# Autodesk Inventor assembly: box
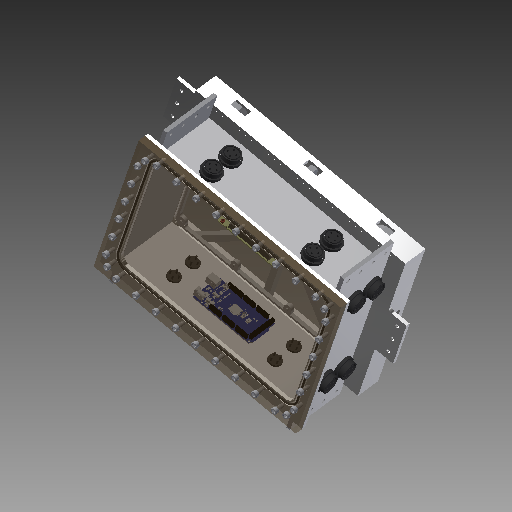
[picture p0: Inventor's stored thumbnail of the model, 512x512]
Saved by Autodesk Inventor 2018.1 (Build 221171000, 171)
## iProperties
Created: 2017-08-02
Part Number: box
Document SubType Name: Assembly
Designer: Kai
Author: Kai
## Documents named in this file (19)
- E:\robosub\box.iam
- E:\robosub\longsides.ipt
- E:\robosub\shortsides.ipt
- E:\robosub\smallgasketback.ipt
- E:\robosub\91292A137_TYPE 18-8 SS SOCKET HEAD CAP SCREW.ipt
- E:\robosub\top.ipt
- E:\robosub\toppoly.ipt
- E:\robosub\bottom3.ipt
- E:\robosub\alumbottom3.ipt
- E:\robosub\pin holder.ipt
- E:\robosub\pins.ipt
- E:\robosub\91292A134_TYPE 18-8 SS SOCKET HEAD CAP SCREW.ipt
- E:\robosub\lid guide.ipt
- E:\robosub\99397A074_METRIC THREAD-FORMING SCREW FOR PLASTICS.ipt
- E:\robosub\latchplate.ipt
- E:\robosub\latchplate2.ipt
- E:\robosub\NUC5i3MYBE- GRABCAD.ipt
- E:\robosub\arduino MEGA2650.ipt
- E:\robosub\connector.ipt
## Components (83 placed, 18 different names)
1. longsides:1 — Mate:6, Flush:8, Mate:242, Mate:252, Mate:253, Mate:254, Mate:255, Mate:256, Mate:257, Mate:258, Mate:259, Mate:260
2. longsides:2 — Mate:3, Mate:106, Mate:107, Mate:108, Mate:109, Flush:3, Flush:20, Mate:240, Mate:248, Mate:249, Mate:250, Mate:251, Mate:261, Mate:262, Mate:263, Mate:264
3. shortsides:1 — Mate:3, Mate:106, Mate:108, Flush:9, Mate:116, Mate:239
4. shortsides:2 — Mate:6, Mate:107, Mate:109, Mate:111, Mate:112, Mate:239, Mate:241, Mate:243, Mate:244, Mate:245, Mate:246, Mate:247, Tangent:2, Tangent:3, Tangent:4, Tangent:5, Tangent:6, Tangent:8
5. smallgasketback:1 — Mate:117, Mate:118
6. top:1 — Mate:111, Mate:112, Flush:3, Mate:113, Mate:114, Mate:115, Flush:4, Flush:5, Mate:213, Mate:214, Mate:235, Flush:12, Flush:13, Mate:236, Flush:14, Flush:15, Mate:237, Flush:16, Mate:238, Flush:18
7. smallgasketback:2 — Mate:113, Mate:114
8. toppoly:1 — Mate:115, Flush:4, Flush:5, Mate:193, Flush:10, Flush:11, Mate:212
9. bottom3:1 — Mate:119, Mate:120, Mate:121, Mate:122, Mate:123, Mate:124, Mate:125, Mate:126, Mate:127, Mate:128, Mate:129, Mate:130, Mate:131, Mate:132, Mate:133, Mate:134, Mate:135, Mate:136, Mate:137, Mate:138, Mate:139, Mate:140, Mate:141, Mate:142, Mate:143, Mate:144, Mate:145, Mate:146, Mate:147, Mate:148, Mate:149, Mate:150, Mate:151, Mate:152, Mate:153, Mate:154, Mate:155, Mate:156, Mate:157, Mate:158, Mate:159, Mate:160, Mate:161, Mate:162, Mate:163, Mate:164, Mate:165, Mate:166, Mate:167, Mate:168, Mate:169, Mate:170, Mate:171, Mate:172, Mate:173, Mate:174, Mate:175, Mate:176, Mate:177, Mate:178, Mate:179, Mate:180, Mate:181, Mate:182, Mate:183, Mate:184, Mate:185, Mate:186, Mate:187, Mate:188, Mate:189
10. alumbottom3:1 — Flush:8, Flush:9, Mate:116, Mate:117, Mate:118, Mate:119, Mate:120, Mate:121, Flush:20, Flush:21, Flush:22, Mate:256
11. 91292A137_TYPE 18-8 SS SOCKET HEAD CAP SCREW:1 — Mate:123, Mate:188
12. 91292A137_TYPE 18-8 SS SOCKET HEAD CAP SCREW:2 — Mate:124, Mate:189
13. 91292A137_TYPE 18-8 SS SOCKET HEAD CAP SCREW:3 — Mate:125, Mate:158
14. 91292A137_TYPE 18-8 SS SOCKET HEAD CAP SCREW:4 — Mate:126, Mate:157
15. 91292A137_TYPE 18-8 SS SOCKET HEAD CAP SCREW:5 — Mate:127, Mate:156
16. 91292A137_TYPE 18-8 SS SOCKET HEAD CAP SCREW:6 — Mate:128, Mate:159
17. 91292A137_TYPE 18-8 SS SOCKET HEAD CAP SCREW:7 — Mate:129, Mate:160
18. 91292A137_TYPE 18-8 SS SOCKET HEAD CAP SCREW:8 — Mate:130, Mate:161
19. 91292A137_TYPE 18-8 SS SOCKET HEAD CAP SCREW:9 — Mate:131, Mate:162
20. 91292A137_TYPE 18-8 SS SOCKET HEAD CAP SCREW:10 — Mate:132, Mate:163
21. 91292A137_TYPE 18-8 SS SOCKET HEAD CAP SCREW:11 — Mate:133, Mate:164
22. 91292A137_TYPE 18-8 SS SOCKET HEAD CAP SCREW:12 — Mate:134, Mate:165
23. 91292A137_TYPE 18-8 SS SOCKET HEAD CAP SCREW:13 — Mate:135, Mate:166
24. 91292A137_TYPE 18-8 SS SOCKET HEAD CAP SCREW:14 — Mate:136, Mate:167
25. 91292A137_TYPE 18-8 SS SOCKET HEAD CAP SCREW:15 — Mate:137, Mate:168
26. 91292A137_TYPE 18-8 SS SOCKET HEAD CAP SCREW:16 — Mate:138, Mate:169
27. 91292A137_TYPE 18-8 SS SOCKET HEAD CAP SCREW:17 — Mate:139, Mate:170
28. 91292A137_TYPE 18-8 SS SOCKET HEAD CAP SCREW:18 — Mate:140, Mate:171
29. 91292A137_TYPE 18-8 SS SOCKET HEAD CAP SCREW:19 — Mate:141, Mate:172
30. 91292A137_TYPE 18-8 SS SOCKET HEAD CAP SCREW:20 — Mate:142, Mate:173
31. 91292A137_TYPE 18-8 SS SOCKET HEAD CAP SCREW:21 — Mate:144, Mate:175
32. 91292A137_TYPE 18-8 SS SOCKET HEAD CAP SCREW:22 — Mate:143, Mate:174
33. 91292A137_TYPE 18-8 SS SOCKET HEAD CAP SCREW:23 — Mate:145, Mate:176
34. 91292A137_TYPE 18-8 SS SOCKET HEAD CAP SCREW:24 — Mate:147, Mate:178
35. 91292A137_TYPE 18-8 SS SOCKET HEAD CAP SCREW:25 — Mate:148, Mate:179
36. 91292A137_TYPE 18-8 SS SOCKET HEAD CAP SCREW:26 — Mate:149, Mate:180
37. 91292A137_TYPE 18-8 SS SOCKET HEAD CAP SCREW:27 — Mate:150, Mate:181
38. 91292A137_TYPE 18-8 SS SOCKET HEAD CAP SCREW:28 — Mate:151, Mate:182
39. 91292A137_TYPE 18-8 SS SOCKET HEAD CAP SCREW:29 — Mate:152, Mate:183
40. 91292A137_TYPE 18-8 SS SOCKET HEAD CAP SCREW:30 — Mate:153, Mate:184
41. 91292A137_TYPE 18-8 SS SOCKET HEAD CAP SCREW:31 — Mate:154, Mate:185
42. 91292A137_TYPE 18-8 SS SOCKET HEAD CAP SCREW:32 — Mate:155, Mate:186
43. 91292A137_TYPE 18-8 SS SOCKET HEAD CAP SCREW:33 — Mate:146, Mate:177
44. 91292A137_TYPE 18-8 SS SOCKET HEAD CAP SCREW:34 — Mate:122, Mate:187
45. pin holder:1 — Mate:194, Mate:195
46. pins:1 — Mate:193, Mate:194, Mate:195, Flush:10, Flush:11, Mate:196, Mate:197, Mate:198, Mate:199, Mate:200, Mate:201, Mate:202, Mate:203, Mate:204, Mate:205, Mate:206, Mate:207, Mate:208, Mate:209, Mate:210, Mate:211
47. 91292A134_TYPE 18-8 SS SOCKET HEAD CAP SCREW:1 — Mate:199, Mate:208
48. 91292A134_TYPE 18-8 SS SOCKET HEAD CAP SCREW:2 — Mate:201, Mate:205
49. 91292A134_TYPE 18-8 SS SOCKET HEAD CAP SCREW:3 — Mate:200, Mate:207
50. 91292A134_TYPE 18-8 SS SOCKET HEAD CAP SCREW:4 — Mate:202, Mate:211
51. 91292A134_TYPE 18-8 SS SOCKET HEAD CAP SCREW:5 — Mate:197, Mate:209
52. 91292A134_TYPE 18-8 SS SOCKET HEAD CAP SCREW:6 — Mate:196, Mate:204
53. 91292A134_TYPE 18-8 SS SOCKET HEAD CAP SCREW:7 — Mate:198, Mate:210
54. 91292A134_TYPE 18-8 SS SOCKET HEAD CAP SCREW:8 — Mate:203, Mate:206
55. lid guide:1 — Mate:212, Mate:213, Mate:214, Mate:215, Mate:216, Mate:217, Mate:218, Mate:219, Mate:220, Mate:221, Mate:222, Mate:223, Mate:224, Mate:225, Mate:226, Mate:227, Mate:228, Mate:229, Mate:230, Mate:231, Mate:232, Mate:233, Mate:234
56. 99397A074_METRIC THREAD-FORMING SCREW FOR PLASTICS:1 — Mate:224, Mate:226
57. 99397A074_METRIC THREAD-FORMING SCREW FOR PLASTICS:2 — Mate:215, Mate:231
58. 99397A074_METRIC THREAD-FORMING SCREW FOR PLASTICS:3 — Mate:221, Mate:228
59. 99397A074_METRIC THREAD-FORMING SCREW FOR PLASTICS:4 — Mate:222, Mate:227
60. 99397A074_METRIC THREAD-FORMING SCREW FOR PLASTICS:5 — Mate:217, Mate:230
61. 99397A074_METRIC THREAD-FORMING SCREW FOR PLASTICS:6 — Mate:216, Mate:232
62. 99397A074_METRIC THREAD-FORMING SCREW FOR PLASTICS:7 — Mate:223, Mate:225
63. 99397A074_METRIC THREAD-FORMING SCREW FOR PLASTICS:8 — Mate:219, Mate:229
64. 99397A074_METRIC THREAD-FORMING SCREW FOR PLASTICS:9 — Mate:218, Mate:233
65. 99397A074_METRIC THREAD-FORMING SCREW FOR PLASTICS:10 — Mate:220, Mate:234
66. latchplate:2 — Mate:235, Flush:12, Flush:13
67. latchplate:3 — Mate:236, Flush:14, Flush:15, Flush:17, Flush:19
68. latchplate2:1 — Mate:237, Flush:16, Flush:17, Tangent:1, Tangent:7
69. latchplate2:2 — Mate:238, Flush:18, Flush:19
70. NUC5i3MYBE- GRABCAD:1 — Mate:240, Flush:21, Mate:241
71. arduino MEGA2650:1 — Mate:242, Flush:22, Mate:243
72. connector:1 — Mate:244, Tangent:1, Tangent:2
73. connector:2 — Mate:245, Tangent:7, Tangent:8
74. connector:3 — Mate:246, Tangent:5, Tangent:6
75. connector:4 — Mate:247, Tangent:3, Tangent:4
76. connector:5 — Mate:248, Mate:262
77. connector:6 — Mate:251, Mate:263
78. connector:7 — Mate:249, Mate:264
79. connector:8 — Mate:250, Mate:261
80. connector:9 — Mate:253, Mate:257
81. connector:10 — Mate:255, Mate:259
82. connector:11 — Mate:252, Mate:258
83. connector:12 — Mate:254, Mate:260
## Relationships (183: Mate 157, Flush 18, Tangent 8)
- Mate:3: longsides:2 ↔ shortsides:1
- Mate:6: longsides:1 ↔ shortsides:2
- Mate:106: longsides:2 ↔ shortsides:1
- Mate:107: longsides:2 ↔ shortsides:2
- Mate:108: longsides:2 ↔ shortsides:1
- Mate:109: longsides:2 ↔ shortsides:2
- Mate:111: shortsides:2 ↔ top:1
- Mate:112 (304.8 mm): shortsides:2 ↔ top:1
- Flush:3 (-19.05 mm): longsides:2 ↔ top:1
- Mate:113: top:1 ↔ smallgasketback:2
- Mate:114: top:1 ↔ smallgasketback:2
- Mate:115: top:1 ↔ toppoly:1
- Flush:4: top:1 ↔ toppoly:1
- Flush:5: top:1 ↔ toppoly:1
- Flush:8: longsides:1 ↔ alumbottom3:1
- Flush:9: shortsides:1 ↔ alumbottom3:1
- Mate:116: shortsides:1 ↔ alumbottom3:1
- Mate:117: smallgasketback:1 ↔ alumbottom3:1
- Mate:118: smallgasketback:1 ↔ alumbottom3:1
- Mate:119: bottom3:1 ↔ alumbottom3:1
- Mate:120: bottom3:1 ↔ alumbottom3:1
- Mate:121: bottom3:1 ↔ alumbottom3:1
- Mate:122: bottom3:1 ↔ 91292A137_TYPE 18-8 SS SOCKET HEAD CAP SCREW:34
- Mate:123: bottom3:1 ↔ 91292A137_TYPE 18-8 SS SOCKET HEAD CAP SCREW:1
- Mate:124: bottom3:1 ↔ 91292A137_TYPE 18-8 SS SOCKET HEAD CAP SCREW:2
- Mate:125: bottom3:1 ↔ 91292A137_TYPE 18-8 SS SOCKET HEAD CAP SCREW:3
- Mate:126: bottom3:1 ↔ 91292A137_TYPE 18-8 SS SOCKET HEAD CAP SCREW:4
- Mate:127: bottom3:1 ↔ 91292A137_TYPE 18-8 SS SOCKET HEAD CAP SCREW:5
- Mate:128: bottom3:1 ↔ 91292A137_TYPE 18-8 SS SOCKET HEAD CAP SCREW:6
- Mate:129: bottom3:1 ↔ 91292A137_TYPE 18-8 SS SOCKET HEAD CAP SCREW:7
- Mate:130: bottom3:1 ↔ 91292A137_TYPE 18-8 SS SOCKET HEAD CAP SCREW:8
- Mate:131: bottom3:1 ↔ 91292A137_TYPE 18-8 SS SOCKET HEAD CAP SCREW:9
- Mate:132: bottom3:1 ↔ 91292A137_TYPE 18-8 SS SOCKET HEAD CAP SCREW:10
- Mate:133: bottom3:1 ↔ 91292A137_TYPE 18-8 SS SOCKET HEAD CAP SCREW:11
- Mate:134: bottom3:1 ↔ 91292A137_TYPE 18-8 SS SOCKET HEAD CAP SCREW:12
- Mate:135: bottom3:1 ↔ 91292A137_TYPE 18-8 SS SOCKET HEAD CAP SCREW:13
- Mate:136: bottom3:1 ↔ 91292A137_TYPE 18-8 SS SOCKET HEAD CAP SCREW:14
- Mate:137: bottom3:1 ↔ 91292A137_TYPE 18-8 SS SOCKET HEAD CAP SCREW:15
- Mate:138: bottom3:1 ↔ 91292A137_TYPE 18-8 SS SOCKET HEAD CAP SCREW:16
- Mate:139: bottom3:1 ↔ 91292A137_TYPE 18-8 SS SOCKET HEAD CAP SCREW:17
- Mate:140: bottom3:1 ↔ 91292A137_TYPE 18-8 SS SOCKET HEAD CAP SCREW:18
- Mate:141: bottom3:1 ↔ 91292A137_TYPE 18-8 SS SOCKET HEAD CAP SCREW:19
- Mate:142: bottom3:1 ↔ 91292A137_TYPE 18-8 SS SOCKET HEAD CAP SCREW:20
- Mate:143: bottom3:1 ↔ 91292A137_TYPE 18-8 SS SOCKET HEAD CAP SCREW:22
- Mate:144: bottom3:1 ↔ 91292A137_TYPE 18-8 SS SOCKET HEAD CAP SCREW:21
- Mate:145: bottom3:1 ↔ 91292A137_TYPE 18-8 SS SOCKET HEAD CAP SCREW:23
- Mate:146: bottom3:1 ↔ 91292A137_TYPE 18-8 SS SOCKET HEAD CAP SCREW:33
- Mate:147: bottom3:1 ↔ 91292A137_TYPE 18-8 SS SOCKET HEAD CAP SCREW:24
- Mate:148: bottom3:1 ↔ 91292A137_TYPE 18-8 SS SOCKET HEAD CAP SCREW:25
- Mate:149: bottom3:1 ↔ 91292A137_TYPE 18-8 SS SOCKET HEAD CAP SCREW:26
- Mate:150: bottom3:1 ↔ 91292A137_TYPE 18-8 SS SOCKET HEAD CAP SCREW:27
- Mate:151: bottom3:1 ↔ 91292A137_TYPE 18-8 SS SOCKET HEAD CAP SCREW:28
- Mate:152: bottom3:1 ↔ 91292A137_TYPE 18-8 SS SOCKET HEAD CAP SCREW:29
- Mate:153: bottom3:1 ↔ 91292A137_TYPE 18-8 SS SOCKET HEAD CAP SCREW:30
- Mate:154: bottom3:1 ↔ 91292A137_TYPE 18-8 SS SOCKET HEAD CAP SCREW:31
- Mate:155: bottom3:1 ↔ 91292A137_TYPE 18-8 SS SOCKET HEAD CAP SCREW:32
- Mate:156: bottom3:1 ↔ 91292A137_TYPE 18-8 SS SOCKET HEAD CAP SCREW:5
- Mate:157: bottom3:1 ↔ 91292A137_TYPE 18-8 SS SOCKET HEAD CAP SCREW:4
- Mate:158: bottom3:1 ↔ 91292A137_TYPE 18-8 SS SOCKET HEAD CAP SCREW:3
- Mate:159: bottom3:1 ↔ 91292A137_TYPE 18-8 SS SOCKET HEAD CAP SCREW:6
- Mate:160: bottom3:1 ↔ 91292A137_TYPE 18-8 SS SOCKET HEAD CAP SCREW:7
- Mate:161: bottom3:1 ↔ 91292A137_TYPE 18-8 SS SOCKET HEAD CAP SCREW:8
- Mate:162: bottom3:1 ↔ 91292A137_TYPE 18-8 SS SOCKET HEAD CAP SCREW:9
- Mate:163: bottom3:1 ↔ 91292A137_TYPE 18-8 SS SOCKET HEAD CAP SCREW:10
- Mate:164: bottom3:1 ↔ 91292A137_TYPE 18-8 SS SOCKET HEAD CAP SCREW:11
- Mate:165: bottom3:1 ↔ 91292A137_TYPE 18-8 SS SOCKET HEAD CAP SCREW:12
- Mate:166: bottom3:1 ↔ 91292A137_TYPE 18-8 SS SOCKET HEAD CAP SCREW:13
- Mate:167: bottom3:1 ↔ 91292A137_TYPE 18-8 SS SOCKET HEAD CAP SCREW:14
- Mate:168: bottom3:1 ↔ 91292A137_TYPE 18-8 SS SOCKET HEAD CAP SCREW:15
- Mate:169: bottom3:1 ↔ 91292A137_TYPE 18-8 SS SOCKET HEAD CAP SCREW:16
- Mate:170: bottom3:1 ↔ 91292A137_TYPE 18-8 SS SOCKET HEAD CAP SCREW:17
- Mate:171: bottom3:1 ↔ 91292A137_TYPE 18-8 SS SOCKET HEAD CAP SCREW:18
- Mate:172: bottom3:1 ↔ 91292A137_TYPE 18-8 SS SOCKET HEAD CAP SCREW:19
- Mate:173: bottom3:1 ↔ 91292A137_TYPE 18-8 SS SOCKET HEAD CAP SCREW:20
- Mate:174: bottom3:1 ↔ 91292A137_TYPE 18-8 SS SOCKET HEAD CAP SCREW:22
- Mate:175: bottom3:1 ↔ 91292A137_TYPE 18-8 SS SOCKET HEAD CAP SCREW:21
- Mate:176: bottom3:1 ↔ 91292A137_TYPE 18-8 SS SOCKET HEAD CAP SCREW:23
- Mate:177: bottom3:1 ↔ 91292A137_TYPE 18-8 SS SOCKET HEAD CAP SCREW:33
- Mate:178: bottom3:1 ↔ 91292A137_TYPE 18-8 SS SOCKET HEAD CAP SCREW:24
- Mate:179: bottom3:1 ↔ 91292A137_TYPE 18-8 SS SOCKET HEAD CAP SCREW:25
- Mate:180: bottom3:1 ↔ 91292A137_TYPE 18-8 SS SOCKET HEAD CAP SCREW:26
- Mate:181: bottom3:1 ↔ 91292A137_TYPE 18-8 SS SOCKET HEAD CAP SCREW:27
- Mate:182: bottom3:1 ↔ 91292A137_TYPE 18-8 SS SOCKET HEAD CAP SCREW:28
- Mate:183: bottom3:1 ↔ 91292A137_TYPE 18-8 SS SOCKET HEAD CAP SCREW:29
- Mate:184: bottom3:1 ↔ 91292A137_TYPE 18-8 SS SOCKET HEAD CAP SCREW:30
- Mate:185: bottom3:1 ↔ 91292A137_TYPE 18-8 SS SOCKET HEAD CAP SCREW:31
- Mate:186: bottom3:1 ↔ 91292A137_TYPE 18-8 SS SOCKET HEAD CAP SCREW:32
- Mate:187: bottom3:1 ↔ 91292A137_TYPE 18-8 SS SOCKET HEAD CAP SCREW:34
- Mate:188: bottom3:1 ↔ 91292A137_TYPE 18-8 SS SOCKET HEAD CAP SCREW:1
- Mate:189: bottom3:1 ↔ 91292A137_TYPE 18-8 SS SOCKET HEAD CAP SCREW:2
- Mate:193: toppoly:1 ↔ pins:1
- Mate:194: pin holder:1 ↔ pins:1
- Mate:195: pin holder:1 ↔ pins:1
- Flush:10 (-6.35 mm): toppoly:1 ↔ pins:1
- Flush:11 (-6.35 mm): toppoly:1 ↔ pins:1
- Mate:196: pins:1 ↔ 91292A134_TYPE 18-8 SS SOCKET HEAD CAP SCREW:6
- Mate:197: pins:1 ↔ 91292A134_TYPE 18-8 SS SOCKET HEAD CAP SCREW:5
- Mate:198: pins:1 ↔ 91292A134_TYPE 18-8 SS SOCKET HEAD CAP SCREW:7
- Mate:199: pins:1 ↔ 91292A134_TYPE 18-8 SS SOCKET HEAD CAP SCREW:1
- Mate:200: pins:1 ↔ 91292A134_TYPE 18-8 SS SOCKET HEAD CAP SCREW:3
- Mate:201: pins:1 ↔ 91292A134_TYPE 18-8 SS SOCKET HEAD CAP SCREW:2
- Mate:202: pins:1 ↔ 91292A134_TYPE 18-8 SS SOCKET HEAD CAP SCREW:4
- Mate:203: pins:1 ↔ 91292A134_TYPE 18-8 SS SOCKET HEAD CAP SCREW:8
- Mate:204: pins:1 ↔ 91292A134_TYPE 18-8 SS SOCKET HEAD CAP SCREW:6
- Mate:205: pins:1 ↔ 91292A134_TYPE 18-8 SS SOCKET HEAD CAP SCREW:2
- Mate:206: pins:1 ↔ 91292A134_TYPE 18-8 SS SOCKET HEAD CAP SCREW:8
- Mate:207: pins:1 ↔ 91292A134_TYPE 18-8 SS SOCKET HEAD CAP SCREW:3
- Mate:208: pins:1 ↔ 91292A134_TYPE 18-8 SS SOCKET HEAD CAP SCREW:1
- Mate:209: pins:1 ↔ 91292A134_TYPE 18-8 SS SOCKET HEAD CAP SCREW:5
- Mate:210: pins:1 ↔ 91292A134_TYPE 18-8 SS SOCKET HEAD CAP SCREW:7
- Mate:211: pins:1 ↔ 91292A134_TYPE 18-8 SS SOCKET HEAD CAP SCREW:4
- Mate:212: toppoly:1 ↔ lid guide:1
- Mate:213: top:1 ↔ lid guide:1
- Mate:214: top:1 ↔ lid guide:1
- Mate:215: lid guide:1 ↔ 99397A074_METRIC THREAD-FORMING SCREW FOR PLASTICS:2
- Mate:216: lid guide:1 ↔ 99397A074_METRIC THREAD-FORMING SCREW FOR PLASTICS:6
- Mate:217: lid guide:1 ↔ 99397A074_METRIC THREAD-FORMING SCREW FOR PLASTICS:5
- Mate:218: lid guide:1 ↔ 99397A074_METRIC THREAD-FORMING SCREW FOR PLASTICS:9
- Mate:219: lid guide:1 ↔ 99397A074_METRIC THREAD-FORMING SCREW FOR PLASTICS:8
- Mate:220: lid guide:1 ↔ 99397A074_METRIC THREAD-FORMING SCREW FOR PLASTICS:10
- Mate:221: lid guide:1 ↔ 99397A074_METRIC THREAD-FORMING SCREW FOR PLASTICS:3
- Mate:222: lid guide:1 ↔ 99397A074_METRIC THREAD-FORMING SCREW FOR PLASTICS:4
- Mate:223: lid guide:1 ↔ 99397A074_METRIC THREAD-FORMING SCREW FOR PLASTICS:7
- Mate:224: lid guide:1 ↔ 99397A074_METRIC THREAD-FORMING SCREW FOR PLASTICS:1
- Mate:225: lid guide:1 ↔ 99397A074_METRIC THREAD-FORMING SCREW FOR PLASTICS:7
- Mate:226: lid guide:1 ↔ 99397A074_METRIC THREAD-FORMING SCREW FOR PLASTICS:1
- Mate:227: lid guide:1 ↔ 99397A074_METRIC THREAD-FORMING SCREW FOR PLASTICS:4
- Mate:228: lid guide:1 ↔ 99397A074_METRIC THREAD-FORMING SCREW FOR PLASTICS:3
- Mate:229: lid guide:1 ↔ 99397A074_METRIC THREAD-FORMING SCREW FOR PLASTICS:8
- Mate:230: lid guide:1 ↔ 99397A074_METRIC THREAD-FORMING SCREW FOR PLASTICS:5
- Mate:231: lid guide:1 ↔ 99397A074_METRIC THREAD-FORMING SCREW FOR PLASTICS:2
- Mate:232: lid guide:1 ↔ 99397A074_METRIC THREAD-FORMING SCREW FOR PLASTICS:6
- Mate:233: lid guide:1 ↔ 99397A074_METRIC THREAD-FORMING SCREW FOR PLASTICS:9
- Mate:234: lid guide:1 ↔ 99397A074_METRIC THREAD-FORMING SCREW FOR PLASTICS:10
- Mate:235: top:1 ↔ latchplate:2
- Flush:12: top:1 ↔ latchplate:2
- Flush:13: top:1 ↔ latchplate:2
- Mate:236: top:1 ↔ latchplate:3
- Flush:14: top:1 ↔ latchplate:3
- Flush:15: top:1 ↔ latchplate:3
- Mate:237: top:1 ↔ latchplate2:1
- Flush:16: top:1 ↔ latchplate2:1
- Flush:17: latchplate:3 ↔ latchplate2:1
- Mate:238: top:1 ↔ latchplate2:2
- Flush:18: top:1 ↔ latchplate2:2
- Flush:19: latchplate:3 ↔ latchplate2:2
- Flush:20: longsides:2 ↔ alumbottom3:1
- Mate:239: shortsides:1 ↔ shortsides:2
- Mate:240 (12.7 mm): longsides:2 ↔ NUC5i3MYBE- GRABCAD:1
- Flush:21 (2.54 mm): alumbottom3:1 ↔ NUC5i3MYBE- GRABCAD:1
- Mate:241 (88.9 mm): shortsides:2 ↔ NUC5i3MYBE- GRABCAD:1
- Mate:242: longsides:1 ↔ arduino MEGA2650:1
- Flush:22 (31.75 mm): alumbottom3:1 ↔ arduino MEGA2650:1
- Mate:243 (101.6 mm): shortsides:2 ↔ arduino MEGA2650:1
- Mate:244: shortsides:2 ↔ connector:1
- Mate:245: shortsides:2 ↔ connector:2
- Mate:246: shortsides:2 ↔ connector:3
- Mate:247: shortsides:2 ↔ connector:4
- Tangent:1 (-76.2 mm): latchplate2:1 ↔ connector:1
- Tangent:2 (-88.9 mm): shortsides:2 ↔ connector:1
- Tangent:3 (-88.9 mm): shortsides:2 ↔ connector:4
- Tangent:4 (-76.2 mm): shortsides:2 ↔ connector:4
- Tangent:5 (-76.2 mm): shortsides:2 ↔ connector:3
- Tangent:6 (-88.9 mm): shortsides:2 ↔ connector:3
- Tangent:7 (-79.375 mm): latchplate2:1 ↔ connector:2
- Tangent:8 (-88.9 mm): shortsides:2 ↔ connector:2
- Mate:248: longsides:2 ↔ connector:5
- Mate:249: longsides:2 ↔ connector:7
- Mate:250: longsides:2 ↔ connector:8
- Mate:251: longsides:2 ↔ connector:6
- Mate:252: longsides:1 ↔ connector:11
- Mate:253: longsides:1 ↔ connector:9
- Mate:254: longsides:1 ↔ connector:12
- Mate:255: longsides:1 ↔ connector:10
- Mate:256: longsides:1 ↔ alumbottom3:1
- Mate:257: longsides:1 ↔ connector:9
- Mate:258: longsides:1 ↔ connector:11
- Mate:259: longsides:1 ↔ connector:10
- Mate:260: longsides:1 ↔ connector:12
- Mate:261: longsides:2 ↔ connector:8
- Mate:262: longsides:2 ↔ connector:5
- Mate:263: longsides:2 ↔ connector:6
- Mate:264: longsides:2 ↔ connector:7
